# Autodesk Inventor assembly: Samenstelling aandrijving
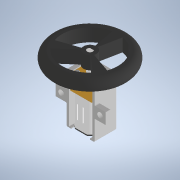
[picture p0: Inventor's stored thumbnail of the model, 180x180]
Saved by Autodesk Inventor 2022 (Build 260153000, 153)
## iProperties
Created: 2022-10-22
Part Number: Samenstelling aandrijving
Document SubType Name: Assembly
Designer: gebruiker
Author: gebruiker
## Documents named in this file (4)
- C:\Users\gebruiker\Documents\Inventor\Linefollower\Samenstelling aandrijving.iam
- C:\Users\gebruiker\Documents\Inventor\Ondersteuning motor.ipt
- C:\Users\gebruiker\Documents\Inventor\Linefollower\Metal gear motor_DC.ipt
- C:\Users\gebruiker\Documents\Inventor\Linefollower\Wiel.ipt
## Components (3 placed, 3 different names)
1. Ondersteuning motor:2 — Flush:2, Mate:3, Mate:4
2. Metal gear motor_DC:2 — Flush:2, Mate:3, Mate:4, Mate:5, Mate:6
3. Wiel:1 — Mate:5, Mate:6
## Relationships (5: Mate 4, Flush 1)
- Flush:2: Ondersteuning motor:2 ↔ Metal gear motor_DC:2
- Mate:3 (0.25 mm): Ondersteuning motor:2 ↔ Metal gear motor_DC:2
- Mate:4: Ondersteuning motor:2 ↔ Metal gear motor_DC:2
- Mate:5: Metal gear motor_DC:2 ↔ Wiel:1
- Mate:6: Metal gear motor_DC:2 ↔ Wiel:1
